# Autodesk Inventor assembly: BACK PLATE ASSEMBLY
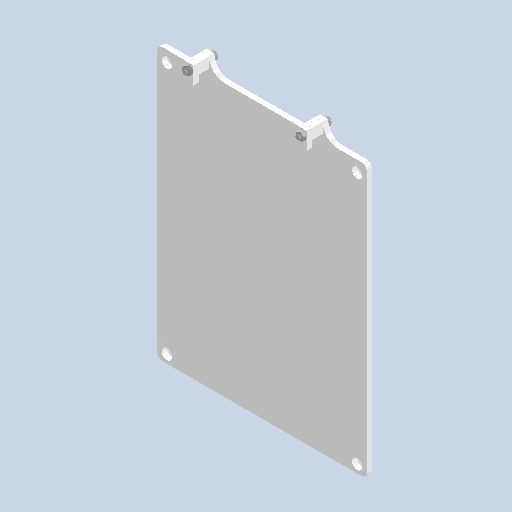
[picture p0: Inventor's stored thumbnail of the model, 512x512]
Saved by Autodesk Inventor 2022 (Build 260153000, 153)
## iProperties
Created: 2021-06-17
Part Number: BACK PLATE ASSEMBLY
Document SubType Name: Assembly
Designer: benka
Author: benka
## Documents named in this file (6)
- C:\Users\benka\Downloads\Sleeker Design\BACK PLATE ASSEMBLY.iam
- C:\Users\benka\Downloads\Sleeker Design\ipt\short back plate spacer.ipt
- C:\Users\benka\Downloads\Sleeker Design\ipt\long back plate spacer.ipt
- C:\Users\benka\Downloads\Sleeker Design\ipt\back plate.ipt
- C:\Users\benka\Downloads\Sleeker Design\ipt\M4 Nut.ipt
- C:\Users\benka\Downloads\Sleeker Design\ipt\M4 Hex Screw v2 - 25.ipt
## Components (11 placed, 5 different names)
1. short back plate spacer:1 — Insert:1, Insert:2, Flush:1, Flush:2
2. short back plate spacer:2 — Insert:2, Mate:1, Flush:2, Mate:4, Flush:3
3. long back plate spacer:1 — Insert:1, Flush:1, Mate:12
4. short back plate spacer:3 — Flush:5, Flush:6
5. short back plate spacer:4 — Mate:2, Mate:3, Flush:4, Flush:5
6. long back plate spacer:2 — Flush:6, Mate:11
7. back plate:1 — Mate:1, Mate:2, Mate:3, Mate:4, Flush:3, Flush:4, Mate:5, Mate:6, Mate:7, Mate:8
8. M4 Hex Screw v2 - 25:1 — Mate:5, Mate:6, Mate:10
9. M4 Hex Screw v2 - 25:2 — Mate:7, Mate:8, Mate:9
10. M4 Nut:1 — Mate:10, Mate:12
11. M4 Nut:2 — Mate:9, Mate:11
## Relationships (22: Mate 12, Flush 6, Insert 4)
- Insert:1: short back plate spacer:1 ↔ long back plate spacer:1
- Insert:2: short back plate spacer:1 ↔ short back plate spacer:2
- [Insert]: short back plate spacer:3 ↔ long back plate spacer:2
- [Insert]: short back plate spacer:3 ↔ short back plate spacer:4
- Mate:1: short back plate spacer:2 ↔ back plate:1
- Mate:2: short back plate spacer:4 ↔ back plate:1
- Mate:3: short back plate spacer:4 ↔ back plate:1
- Flush:1: short back plate spacer:1 ↔ long back plate spacer:1
- Flush:2: short back plate spacer:1 ↔ short back plate spacer:2
- Mate:4: short back plate spacer:2 ↔ back plate:1
- Flush:3: short back plate spacer:2 ↔ back plate:1
- Flush:4: short back plate spacer:4 ↔ back plate:1
- Flush:5: short back plate spacer:3 ↔ short back plate spacer:4
- Flush:6: short back plate spacer:3 ↔ long back plate spacer:2
- Mate:5: back plate:1 ↔ M4 Hex Screw v2 - 25:1
- Mate:6: back plate:1 ↔ M4 Hex Screw v2 - 25:1
- Mate:7: back plate:1 ↔ M4 Hex Screw v2 - 25:2
- Mate:8: back plate:1 ↔ M4 Hex Screw v2 - 25:2
- Mate:9: M4 Hex Screw v2 - 25:2 ↔ M4 Nut:2
- Mate:10: M4 Hex Screw v2 - 25:1 ↔ M4 Nut:1
- Mate:11: long back plate spacer:2 ↔ M4 Nut:2
- Mate:12: long back plate spacer:1 ↔ M4 Nut:1
## Named parameters: d2_d0 = 0 mm, d3_d1 = 0 mm
